# Autodesk Inventor assembly: use this - gimme that tech award
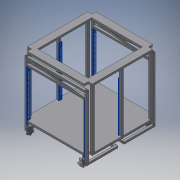
[picture p0: Inventor's stored thumbnail of the model, 180x180]
Saved by Autodesk Inventor 2018 (Build 220112000, 112)
## iProperties
Created: 2019-01-10
Part Number: use this - gimme that tech award
Document SubType Name: Assembly
Designer: maste
Author: maste
## Documents named in this file (6)
- C:\Users\maste\OneDrive\Documents\GitHub\2019CAD\Drivebase but Calvin is a mad man\use this - gimme that tech award.iam
- C:\Users\maste\OneDrive\Documents\GitHub\2019CAD\Drivebase but Calvin is a mad man\Slidey Mecanum L thing.iam
- C:\Users\maste\OneDrive\Documents\GitHub\2019CAD\Drivebase but Calvin is a mad man\Lower Platform.ipt
- C:\Users\maste\OneDrive\Documents\GitHub\2019CAD\Drivebase but Calvin is a mad man\1x1 28 in.ipt
- C:\Users\maste\OneDrive\Documents\GitHub\2019CAD\Drivebase but Calvin is a mad man\User Library-plastic bearings_igus nk02-40-2-610.iam
- C:\Users\maste\OneDrive\Documents\GitHub\2019CAD\Drivebase but Calvin is a mad man\Upper Platform.ipt
## Components (12 placed, 5 different names)
1. Slidey Mecanum L thing:1 [sub-assembly] — Mate:2, Flush:2, Flush:3
2. Slidey Mecanum L thing:2 [sub-assembly] — Mate:1, Flush:1, Flush:3, Mate:3
3. Lower Platform:1 — Mate:1, Flush:1, Mate:2, Flush:2, Mate:3, Flush:4, Flush:5, Mate:4, Mate:5, Flush:6, Flush:7, Flush:8, Flush:9, Mate:6, Flush:10, Flush:11, Mate:7, Flush:12, Mate:8, Flush:13, Mate:9, Flush:14, Flush:15, Mate:11, Mate:13
4. 1x1 28 in:1 — Mate:5, Flush:6, Flush:7
5. 1x1 28 in:2 — Flush:10, Flush:11, Mate:7
6. 1x1 28 in:3 — Flush:4, Flush:5, Mate:4, Mate:14, Mate:15, Mate:16
7. 1x1 28 in:4 — Flush:8, Flush:9, Mate:6
8. 1x1 28 in:5 — Flush:12, Mate:8, Flush:13, Mate:12, Flush:17
9. 1x1 28 in:6 — Mate:9, Flush:14, Flush:15, Mate:10, Flush:16
10. User Library-plastic bearings_igus nk02-40-2-610:1 [sub-assembly] — Mate:10, Mate:11, Flush:16
11. User Library-plastic bearings_igus nk02-40-2-610:2 [sub-assembly] — Mate:12, Mate:13, Flush:17
12. Upper Platform:1 — Mate:14, Mate:15, Mate:16
## Relationships (33: Flush 17, Mate 16)
- Mate:1: Slidey Mecanum L thing:2 ↔ Lower Platform:1
- Flush:1: Slidey Mecanum L thing:2 ↔ Lower Platform:1
- Mate:2: Slidey Mecanum L thing:1 ↔ Lower Platform:1
- Flush:2: Slidey Mecanum L thing:1 ↔ Lower Platform:1
- Flush:3: Slidey Mecanum L thing:1 ↔ Slidey Mecanum L thing:2
- Mate:3 (64.2112 mm): Slidey Mecanum L thing:2 ↔ Lower Platform:1
- Flush:4: Lower Platform:1 ↔ 1x1 28 in:3
- Flush:5: Lower Platform:1 ↔ 1x1 28 in:3
- Mate:4: Lower Platform:1 ↔ 1x1 28 in:3
- Mate:5: Lower Platform:1 ↔ 1x1 28 in:1
- Flush:6: Lower Platform:1 ↔ 1x1 28 in:1
- Flush:7: Lower Platform:1 ↔ 1x1 28 in:1
- Flush:8: Lower Platform:1 ↔ 1x1 28 in:4
- Flush:9: Lower Platform:1 ↔ 1x1 28 in:4
- Mate:6: Lower Platform:1 ↔ 1x1 28 in:4
- Flush:10: Lower Platform:1 ↔ 1x1 28 in:2
- Flush:11: Lower Platform:1 ↔ 1x1 28 in:2
- Mate:7: Lower Platform:1 ↔ 1x1 28 in:2
- Flush:12: Lower Platform:1 ↔ 1x1 28 in:5
- Mate:8: Lower Platform:1 ↔ 1x1 28 in:5
- Flush:13 (355.6 mm): Lower Platform:1 ↔ 1x1 28 in:5
- Mate:9: Lower Platform:1 ↔ 1x1 28 in:6
- Flush:14: Lower Platform:1 ↔ 1x1 28 in:6
- Flush:15 (355.6 mm): Lower Platform:1 ↔ 1x1 28 in:6
- Mate:10: 1x1 28 in:6 ↔ User Library-plastic bearings_igus nk02-40-2-610:1
- Mate:11: Lower Platform:1 ↔ User Library-plastic bearings_igus nk02-40-2-610:1
- Flush:16 (-10.0012 mm): 1x1 28 in:6 ↔ User Library-plastic bearings_igus nk02-40-2-610:1
- Mate:12: 1x1 28 in:5 ↔ User Library-plastic bearings_igus nk02-40-2-610:2
- Mate:13: Lower Platform:1 ↔ User Library-plastic bearings_igus nk02-40-2-610:2
- Flush:17 (-10.0012 mm): 1x1 28 in:5 ↔ User Library-plastic bearings_igus nk02-40-2-610:2
- Mate:14: 1x1 28 in:3 ↔ Upper Platform:1
- Mate:15: 1x1 28 in:3 ↔ Upper Platform:1
- Mate:16: 1x1 28 in:3 ↔ Upper Platform:1
